# Autodesk Inventor assembly: Assembly2 стойка
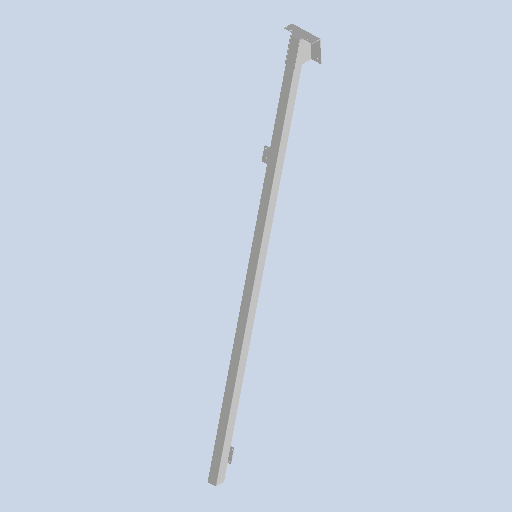
[picture p0: Inventor's stored thumbnail of the model, 512x512]
Saved by Autodesk Inventor 2025 (Build 290162010, 162A)
## iProperties
Created: 2024-06-18
Part Number: Assembly2 стойка
Document SubType Name: Assembly
Designer: admin
Author: admin
## Documents named in this file (7)
- C:\Users\pokla\Documents\Inventor\Goat\Goat-main\Assembly2 стойка.iam
- C:\Users\pokla\Documents\Inventor\Goat\Goat-main\Сrane plate 3.ipt
- C:\Users\pokla\Documents\Inventor\Goat\Goat-main\стойка 1 100x100x4 - 5000.ipt
- C:\Users\pokla\Documents\Inventor\Goat\Goat-main\Сrane plate 4.ipt
- C:\Users\pokla\Documents\Inventor\Goat\Goat-main\Сrane plate 6.ipt
- C:\Users\pokla\Documents\Inventor\Goat\Goat-main\Сrane plate 2.ipt
- C:\Users\pokla\Documents\Inventor\Goat\Goat-main\Сrane plate 5.ipt
## Components (7 placed, 6 different names)
1. Сrane plate 3.ipt:1 — Mate:11, Mate:12, Mate:13
2. стойка 1 100x100x4 - 5000.ipt:1 — Mate:10
3. Сrane plate 4.ipt:1
4. Сrane plate 6.ipt:1
5. Сrane plate 4.ipt:2
6. Сrane plate 2.ipt:1 — Mate:11, Mate:12, Mate:13
7. Сrane plate 5.ipt:1 — Mate:10
## Relationships (18: Mate 13, Flush 5)
- [Mate]: стойка 1 100x100x4 - 5000.ipt:1 ↔ Сrane plate 4.ipt:1
- [Mate]: стойка 1 100x100x4 - 5000.ipt:1 ↔ Сrane plate 4.ipt:2
- [Flush]: стойка 1 100x100x4 - 5000.ipt:1 ↔ Сrane plate 4.ipt:2
- [Flush]: стойка 1 100x100x4 - 5000.ipt:1 ↔ Сrane plate 4.ipt:1
- [Flush]: стойка 1 100x100x4 - 5000.ipt:1 ↔ Сrane plate 4.ipt:1
- [Flush]: стойка 1 100x100x4 - 5000.ipt:1 ↔ Сrane plate 4.ipt:2
- [Flush]: стойка 1 100x100x4 - 5000.ipt:1 ↔ Сrane plate 2.ipt:1
- [Mate]: стойка 1 100x100x4 - 5000.ipt:1 ↔ Сrane plate 2.ipt:1
- [Mate]: стойка 1 100x100x4 - 5000.ipt:1 ↔ Сrane plate 6.ipt:1
- [Mate]: стойка 1 100x100x4 - 5000.ipt:1 ↔ Сrane plate 6.ipt:1
- [Mate]: Сrane plate 3.ipt:1 ↔ Сrane plate 4.ipt:2
- [Mate] (-200 mm): стойка 1 100x100x4 - 5000.ipt:1 ↔ Сrane plate 6.ipt:1
- [Mate]: стойка 1 100x100x4 - 5000.ipt:1 ↔ Сrane plate 5.ipt:1
- [Mate]: стойка 1 100x100x4 - 5000.ipt:1 ↔ Сrane plate 5.ipt:1
- Mate:10 (1280 mm): стойка 1 100x100x4 - 5000.ipt:1 ↔ Сrane plate 5.ipt:1
- Mate:11: Сrane plate 3.ipt:1 ↔ Сrane plate 2.ipt:1
- Mate:12: Сrane plate 3.ipt:1 ↔ Сrane plate 2.ipt:1
- Mate:13: Сrane plate 3.ipt:1 ↔ Сrane plate 2.ipt:1
